# Autodesk Inventor assembly: AC254-080-OnPost
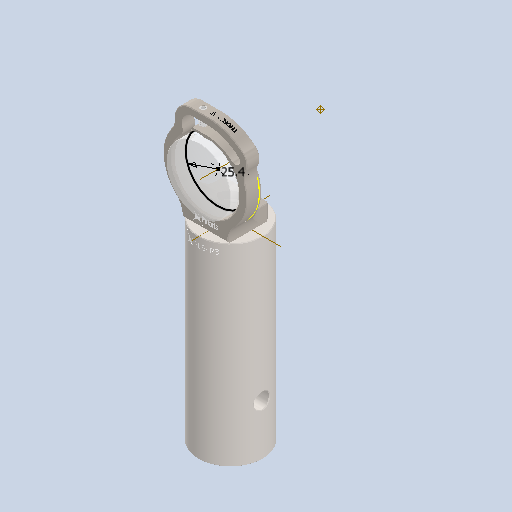
[picture p0: Inventor's stored thumbnail of the model, 512x512]
Saved by Autodesk Inventor 2025.2 (Build 292293000, 293)
## iProperties
Created: 2024-01-26
Part Number: AC254-080-OnPost
Document SubType Name: Assembly
Designer: monolithic
Author: monolithic
## Documents named in this file (3)
- C:\Users\monolithic\Documents\GitHub\CAD\Monolith\John\Altair_PowellBaseplate_SPIM_ASLM_CTASLM\Assembly\SubAssemblies\AC254-080-OnPost.iam
- C:\Users\monolithic\Documents\GitHub\CAD\Monolith\John\Altair_PowellBaseplate_SPIM_ASLM_CTASLM\Assembly\SubAssemblies\PostLensHolder_B1S_PLS3in.iam
- C:\Users\monolithic\Documents\GitHub\CAD\Monolith\John\Altair_PowellBaseplate_SPIM_ASLM_CTASLM\Assembly\SubAssemblies\AC254-080-A-ML.ipt
## Components (2 placed, 2 different names)
1. PostLensHolder_B1S_PLS3in:1 [sub-assembly] — Angle:1, Insert:1, Angle:2, Mate:2, Angle:3
2. AC254-080-A-ML:1 — Angle:1, Insert:1, Mate:1, Tangent:1
## Relationships (7: Angle 3, Mate 2, Insert 1, Tangent 1)
- Angle:1 (-90 deg): PostLensHolder_B1S_PLS3in:1 ↔ AC254-080-A-ML:1
- Insert:1: PostLensHolder_B1S_PLS3in:1 ↔ AC254-080-A-ML:1
- Mate:1: AC254-080-A-ML:1
- Angle:2 (0 deg): PostLensHolder_B1S_PLS3in:1
- Tangent:1: AC254-080-A-ML:1
- Mate:2: PostLensHolder_B1S_PLS3in:1
- Angle:3 (0 deg): PostLensHolder_B1S_PLS3in:1
